# Autodesk Inventor assembly: ClawGen2Prototype
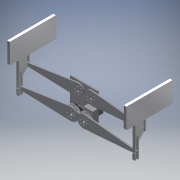
[picture p0: Inventor's stored thumbnail of the model, 180x180]
Saved by Autodesk Inventor 2017 (Build 210142000, 142)
## iProperties
Created: 2017-10-31
Part Number: ClawGen2Prototype
Document SubType Name: Assembly
Designer: User
Author: User
## Documents named in this file (6)
- C:\Robotics\CAD\2017-18_CAD\ClawGen2Prototype.iam
- C:\Robotics\CAD\2017-18_CAD\ClawLinkage.ipt
- C:\Robotics\CAD\2017-18_CAD\ClawServoHolder.ipt
- C:\Robotics\CAD\COTSParts\Tetrix\Tetrix servo 180.ipt
- C:\Robotics\CAD\2017-18_CAD\2BarClawPaddle.ipt
- C:\Robotics\CAD\COTSParts\Tetrix\Tetrix Gear 40T.ipt
## Components (10 placed, 5 different names)
1. ClawLinkage:1 — Mate:7, Mate:16, Mate:17, Mate:21, Insert:2
2. ClawLinkage:2 — Mate:4, Mate:10, Insert:1, Insert:5
3. ClawLinkage:3 — Mate:8, Mate:9, Insert:3
4. ClawLinkage:4 — Mate:6, Mate:15, Mate:18, Insert:4, Mate:22
5. ClawServoHolder:1 — Mate:1, Mate:2, Mate:3, Mate:4, Mate:6, Mate:8, Mate:9, Mate:10, Mate:13, Insert:5
6. Tetrix servo 180:1 — Mate:1, Mate:2, Mate:3, Mate:7
7. 2BarClawPaddle:1 — Mate:18, Insert:3, Insert:4
8. 2BarClawPaddle:2 — Mate:21, Insert:1, Insert:2
9. Tetrix Gear 40T:1 — Mate:13, Mate:15, Mate:22
10. Tetrix Gear 40T:2 — Mate:16, Mate:17
## Relationships (21: Mate 16, Insert 5)
- Mate:1: ClawServoHolder:1 ↔ Tetrix servo 180:1
- Mate:2: ClawServoHolder:1 ↔ Tetrix servo 180:1
- Mate:3: ClawServoHolder:1 ↔ Tetrix servo 180:1
- Mate:4: ClawLinkage:2 ↔ ClawServoHolder:1
- Mate:6: ClawLinkage:4 ↔ ClawServoHolder:1
- Mate:7: ClawLinkage:1 ↔ Tetrix servo 180:1
- Mate:8: ClawLinkage:3 ↔ ClawServoHolder:1
- Mate:9: ClawLinkage:3 ↔ ClawServoHolder:1
- Mate:10: ClawLinkage:2 ↔ ClawServoHolder:1
- Mate:13: ClawServoHolder:1 ↔ Tetrix Gear 40T:1
- Mate:15: ClawLinkage:4 ↔ Tetrix Gear 40T:1
- Mate:16: ClawLinkage:1 ↔ Tetrix Gear 40T:2
- Mate:17: ClawLinkage:1 ↔ Tetrix Gear 40T:2
- Mate:18: ClawLinkage:4 ↔ 2BarClawPaddle:1
- Mate:21: ClawLinkage:1 ↔ 2BarClawPaddle:2
- Insert:1: ClawLinkage:2 ↔ 2BarClawPaddle:2
- Insert:2: ClawLinkage:1 ↔ 2BarClawPaddle:2
- Insert:3: ClawLinkage:3 ↔ 2BarClawPaddle:1
- Insert:4: ClawLinkage:4 ↔ 2BarClawPaddle:1
- Mate:22: ClawLinkage:4 ↔ Tetrix Gear 40T:1
- Insert:5: ClawLinkage:2 ↔ ClawServoHolder:1
